# Autodesk Inventor assembly: 3_25_Omni-Directional_Wheel_217-4775
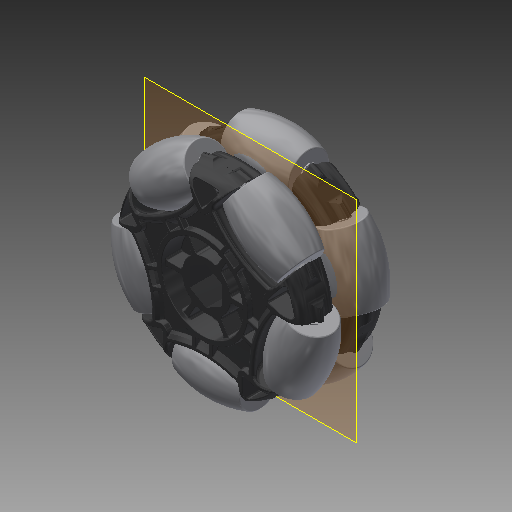
[picture p0: Inventor's stored thumbnail of the model, 512x512]
Saved by Autodesk Inventor 2018.3 (Build 223284000, 284)
## iProperties
Created: 2015-10-21
Part Number: 3_25_Omni-Directional_Wheel_217-4775
Description: STEP AP214
Document SubType Name: Assembly
Designer: user
Sending System: SolidWorks 2015
Preprocessor: SwSTEP 2.0
Title: 217-4775-STEP-20151021.STEP
Revision Number: ANY
## Documents named in this file (8)
- C:\Users\22turnmaxw\Documents\GrabCAD\Infinite Recharge 2020\Build season\3 inch OmniWheel STEP\3_25_Omni-Directional_Wheel_217-4775.iam
- C:\Users\22turnmaxw\Documents\GrabCAD\Infinite Recharge 2020\Build season\3 inch OmniWheel STEP\217-4775-001 Rev5.ipt
- C:\Users\22turnmaxw\Documents\GrabCAD\Infinite Recharge 2020\Build season\3 inch OmniWheel STEP\217-4775-003 Rev5.ipt
- C:\Users\22turnmaxw\Documents\GrabCAD\Infinite Recharge 2020\Build season\3 inch OmniWheel STEP\217-4775-004 Rev1_Smooth.ipt
- C:\Users\22turnmaxw\Documents\GrabCAD\Infinite Recharge 2020\Build season\3 inch OmniWheel STEP\217-4775-005 Rev1.ipt
- C:\Users\22turnmaxw\Documents\GrabCAD\Infinite Recharge 2020\Build season\3 inch OmniWheel STEP\217-4775-007 Rev1.ipt
- C:\Users\22turnmaxw\Documents\GrabCAD\Infinite Recharge 2020\Build season\3 inch OmniWheel STEP\217-2584-009 Rev1.ipt
- C:\Users\22turnmaxw\Documents\GrabCAD\Infinite Recharge 2020\Build season\3 inch OmniWheel STEP\217-2584-007 Rev1_90116A020.ipt
## Components (63 placed, 63 different names)
1. 217-4775-001 Rev5_1
2. 217-4775-003 Rev5_2 — Symmetry:1, Mate:1
3. 217-4775-004 Rev1_Smooth_3
4. 217-4775-004 Rev1_Smooth_4
5. 217-4775-005 Rev1_5
6. 217-4775-005 Rev1_6
7. 217-4775-005 Rev1_7
8. 217-4775-005 Rev1_8
9. 217-4775-005 Rev1_9
10. 217-4775-005 Rev1_10
11. 217-4775-004 Rev1_Smooth_11
12. 217-4775-004 Rev1_Smooth_12
13. 217-4775-004 Rev1_Smooth_13
14. 217-4775-004 Rev1_Smooth_14
15. 217-4775-005 Rev1_15
16. 217-4775-005 Rev1_16
17. 217-4775-005 Rev1_17
18. 217-4775-005 Rev1_18
19. 217-4775-004 Rev1_Smooth_19
20. 217-4775-004 Rev1_Smooth_20
21. 217-4775-004 Rev1_Smooth_21
22. 217-4775-004 Rev1_Smooth_22
23. 217-4775-007 Rev1_23
24. 217-4775-007 Rev1_24
25. 217-4775-007 Rev1_25
26. 217-4775-007 Rev1_26
27. 217-4775-007 Rev1_27
28. 217-4775-007 Rev1_28
29. 217-4775-007 Rev1_29
30. 217-4775-007 Rev1_30
31. 217-4775-007 Rev1_31
32. 217-4775-007 Rev1_32
33. 217-4775-003 Rev5_33 — Symmetry:1
34. 217-2584-009 Rev1_34
35. 217-2584-009 Rev1_35
36. 217-2584-009 Rev1_36
37. 217-2584-009 Rev1_37
38. 217-2584-009 Rev1_38
39. 217-2584-009 Rev1_39
40. 217-2584-009 Rev1_40
41. 217-2584-009 Rev1_41
42. 217-2584-009 Rev1_42
43. 217-2584-009 Rev1_43
44. 217-2584-009 Rev1_44
45. 217-2584-009 Rev1_45
46. 217-2584-009 Rev1_46
47. 217-2584-009 Rev1_47
48. 217-2584-009 Rev1_48
49. 217-2584-009 Rev1_49
50. 217-2584-009 Rev1_50
51. 217-2584-009 Rev1_51
52. 217-2584-009 Rev1_52
53. 217-2584-009 Rev1_53
54. 217-2584-007 Rev1_90116A020_54
55. 217-2584-007 Rev1_90116A020_55
56. 217-2584-007 Rev1_90116A020_56
57. 217-2584-007 Rev1_90116A020_57
58. 217-2584-007 Rev1_90116A020_58
59. 217-2584-007 Rev1_90116A020_59
60. 217-2584-007 Rev1_90116A020_60
61. 217-2584-007 Rev1_90116A020_61
62. 217-2584-007 Rev1_90116A020_62
63. 217-2584-007 Rev1_90116A020_63
## Relationships (2: Symmetry 1, Mate 1)
- Symmetry:1: 217-4775-003 Rev5_2 ↔ 217-4775-003 Rev5_33
- Mate:1: 217-4775-003 Rev5_2
